# Autodesk Inventor assembly: Düse1
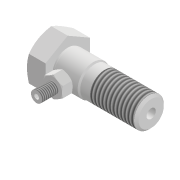
[picture p0: Inventor's stored thumbnail of the model, 180x180]
Saved by Autodesk Inventor 2021 (Build 250183000, 183)
## iProperties
Created: 2021-07-20
Part Number: Düse1
Document SubType Name: Assembly
Designer: lukas
Author: lukas
## Documents named in this file (4)
- C:\Users\lukas\OneDrive - HTBLA Kaindorf\Diplomarbeit\Mechanik\InventorKonstruktion\Düse1.iam
- C:\Users\lukas\OneDrive - HTBLA Kaindorf\Diplomarbeit\Mechanik\InventorKonstruktion\In\de-DE\CNS 4364\CNS 4364 - M16 x 2 x 45.ipt
- C:\Users\lukas\OneDrive - HTBLA Kaindorf\Diplomarbeit\Mechanik\InventorKonstruktion\DüseGewinde.ipt
- C:\Users\lukas\OneDrive - HTBLA Kaindorf\Diplomarbeit\Mechanik\InventorKonstruktion\In\de-DE\ANSI B18.2.4.2M\ANSI B18.2.4.2M - M6x1 - 10.ipt
## Components (3 placed, 3 different names)
1. CNS 4364 M16 x 45:1 — Starr:1
2. DüseGewinde:1 — Starr:1, Drehbar:1
3. ANSI B18.2.4.2M M6x1:1 — Drehbar:1
## Relationships (2: WeldJoint 1, RevoluteJoint 1)
- Starr:1 [WeldJoint] (-5.5 mm): CNS 4364 M16 x 45:1 ↔ DüseGewinde:1
- Drehbar:1 [RevoluteJoint] (-9.25 mm): DüseGewinde:1 ↔ ANSI B18.2.4.2M M6x1:1
